# Autodesk Inventor assembly: motorassembly
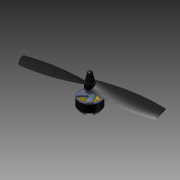
[picture p0: Inventor's stored thumbnail of the model, 180x180]
Saved by Autodesk Inventor 2012 (Build 160160000, 160)
## iProperties
Created: 2014-07-10
Part Number: motorassembly
Document SubType Name: Assembly
Designer: Anon
Author: Anon
## Documents named in this file (4)
- D:\Dropbox\Courses\GP\git\dronestructure\motor\motorassembly.iam
- D:\Dropbox\Courses\GP\git\dronestructure\motor\bldc.iam
- D:\Dropbox\Courses\GP\git\dronestructure\motor\prop.ipt
- D:\Dropbox\Courses\GP\git\dronestructure\motor\nut.ipt
## Components (3 placed, 3 different names)
1. bldc:1 [sub-assembly] — Mate:1, Mate:2, Mate:3
2. prop:1 — Mate:1, Mate:2, Mate:4
3. nut:1 — Mate:3, Mate:4
## Relationships (4: Mate 4)
- Mate:1: bldc:1 ↔ prop:1
- Mate:2: bldc:1 ↔ prop:1
- Mate:3: bldc:1 ↔ nut:1
- Mate:4: prop:1 ↔ nut:1
